# Autodesk Inventor assembly: foot2
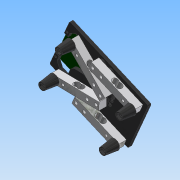
[picture p0: Inventor's stored thumbnail of the model, 180x180]
Saved by Autodesk Inventor 2015 (Build 190159000, 159)
## iProperties
Created: 2015-06-16
Part Number: foot2
Document SubType Name: Assembly
Designer: Gregwar
Author: Gregwar
## Documents named in this file (5)
- C:\Users\Gregwar\Desktop\Meca\SigmabanFoot\foot2.iam
- C:\Users\Gregwar\Desktop\Meca\SigmabanFoot\fix3.ipt
- C:\Users\Gregwar\Desktop\Meca\SigmabanFoot\gauge.ipt
- C:\Users\Gregwar\Desktop\Meca\SigmabanFoot\crampon.ipt
- C:\Users\Gregwar\Desktop\Meca\SigmabanFoot\board.ipt
## Components (10 placed, 4 different names)
1. fix3:1 — Placage:1, Placage:2, Placage:3, Placage:4, Placage:5, Placage:6, Placage:7, Placage:8, Placage:9, Placage:10, Placage:11, Placage:12, Placage:21, Placage:22, Placage:23
2. gauge:1 — Placage:1, Placage:2, Placage:3, Placage:17, Placage:18
3. gauge:2 — Placage:7, Placage:8, Placage:9, Placage:15, Placage:16
4. gauge:3 — Placage:4, Placage:5, Placage:6, Placage:13, Placage:14
5. gauge:4 — Placage:10, Placage:11, Placage:12, Placage:19, Placage:20
6. crampon:1 — Placage:13, Placage:14
7. crampon:2 — Placage:17, Placage:18
8. crampon:3 — Placage:19, Placage:20
9. crampon:4 — Placage:15, Placage:16
10. board:1 — Placage:21, Placage:22, Placage:23
## Relationships (23: Mate 23)
- Placage:1 [Mate]: fix3:1 ↔ gauge:1
- Placage:2 [Mate]: fix3:1 ↔ gauge:1
- Placage:3 [Mate]: fix3:1 ↔ gauge:1
- Placage:4 [Mate]: fix3:1 ↔ gauge:3
- Placage:5 [Mate]: fix3:1 ↔ gauge:3
- Placage:6 [Mate]: fix3:1 ↔ gauge:3
- Placage:7 [Mate]: fix3:1 ↔ gauge:2
- Placage:8 [Mate]: fix3:1 ↔ gauge:2
- Placage:9 [Mate]: fix3:1 ↔ gauge:2
- Placage:10 [Mate]: fix3:1 ↔ gauge:4
- Placage:11 [Mate]: fix3:1 ↔ gauge:4
- Placage:12 [Mate]: fix3:1 ↔ gauge:4
- Placage:13 [Mate]: gauge:3 ↔ crampon:1
- Placage:14 [Mate]: gauge:3 ↔ crampon:1
- Placage:15 [Mate]: gauge:2 ↔ crampon:4
- Placage:16 [Mate]: gauge:2 ↔ crampon:4
- Placage:17 [Mate]: gauge:1 ↔ crampon:2
- Placage:18 [Mate]: gauge:1 ↔ crampon:2
- Placage:19 [Mate]: gauge:4 ↔ crampon:3
- Placage:20 [Mate]: gauge:4 ↔ crampon:3
- Placage:21 [Mate]: fix3:1 ↔ board:1
- Placage:22 [Mate]: fix3:1 ↔ board:1
- Placage:23 [Mate]: fix3:1 ↔ board:1
